# Autodesk Inventor assembly: populated-keyboard_cherrymx
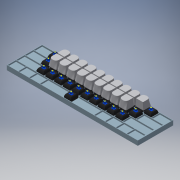
[picture p0: Inventor's stored thumbnail of the model, 180x180]
Saved by Autodesk Inventor 2016 (Build 200138000, 138)
## iProperties
Created: 2016-12-08
Part Number: populated-keyboard_cherrymx
Document SubType Name: Assembly
Designer: Cemra JC
Author: Cemra JC
## Documents named in this file (4)
- J:\The Files\The Software Files\Projects\stenotoppers\cherrymx\base-model\populated-keyboard_cherrymx.iam
- J:\The Files\The Software Files\Projects\stenotoppers\cherrymx\base-model\keyboard-mockup_cherrymx.iam
- J:\The Files\The Software Files\Projects\stenotoppers\cherrymx\base-model\standard-keycap_top-rows_base_cherrymx.ipt
- J:\The Files\The Software Files\Projects\stenotoppers\cherrymx\base-model\keyswitch_cherrymx.iam
## Components (21 placed, 3 different names)
1. keyboard-mockup_cherrymx:1 [sub-assembly] — Rigid:3, Rigid:4, Rigid:5
2. keyswitch_cherrymx:1 [sub-assembly] — Rigid:5
3. standard-keycap_top-rows_base_cherrymx:4 — Rigid:3
4. standard-keycap_top-rows_base_cherrymx:5
5. standard-keycap_top-rows_base_cherrymx:6
6. standard-keycap_top-rows_base_cherrymx:7
7. standard-keycap_top-rows_base_cherrymx:8
8. standard-keycap_top-rows_base_cherrymx:9
9. standard-keycap_top-rows_base_cherrymx:10
10. standard-keycap_top-rows_base_cherrymx:11
11. standard-keycap_top-rows_base_cherrymx:12
12. standard-keycap_top-rows_base_cherrymx:13
13. standard-keycap_top-rows_base_cherrymx:2 — Rigid:4
14. standard-keycap_top-rows_base_cherrymx:14
15. standard-keycap_top-rows_base_cherrymx:15
16. standard-keycap_top-rows_base_cherrymx:16
17. standard-keycap_top-rows_base_cherrymx:17
18. standard-keycap_top-rows_base_cherrymx:18
19. standard-keycap_top-rows_base_cherrymx:19
20. standard-keycap_top-rows_base_cherrymx:20
21. standard-keycap_top-rows_base_cherrymx:21
## Component patterns: (10 elements, first: standard-keycap_top-rows_base_cherrymx:4), (9 elements, first: standard-keycap_top-rows_base_cherrymx:2)
## Relationships (3: WeldJoint 3)
- Rigid:3 [WeldJoint]: keyboard-mockup_cherrymx:1 ↔ standard-keycap_top-rows_base_cherrymx:4
- Rigid:4 [WeldJoint]: keyboard-mockup_cherrymx:1 ↔ standard-keycap_top-rows_base_cherrymx:2
- Rigid:5 [WeldJoint]: keyboard-mockup_cherrymx:1 ↔ keyswitch_cherrymx:1
